# Autodesk Inventor assembly: bubble-wall
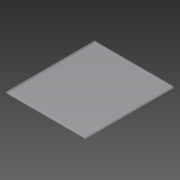
[picture p0: Inventor's stored thumbnail of the model, 180x180]
Saved by Autodesk Inventor 2013 (Build 170138000, 138)
## iProperties
Created: 2013-04-28
Part Number: bubble-wall
Document SubType Name: Assembly
Designer: Chris
Author: Chris
## Documents named in this file (3)
- C:\Users\Chris\Documents\Inventor\Redbull-2013\bubble-wall-final\bubble-wall.iam
- C:\Users\Chris\Documents\Inventor\Redbull-2013\bubble-wall-final\wall-side.ipt
- C:\Users\Chris\Documents\Inventor\Redbull-2013\bubble-wall-final\bottom.ipt
## Components (3 placed, 2 different names)
1. wall-side:1 — Mate:1, Mate:2, Flush:1, Mate:3
2. wall-side:2 — Mate:1, Mate:2, Flush:1, Flush:2, Flush:3
3. bottom:1 — Mate:3, Flush:2, Flush:3
## Relationships (6: Mate 3, Flush 3)
- Mate:1: wall-side:1 ↔ wall-side:2
- Mate:2: wall-side:1 ↔ wall-side:2
- Flush:1: wall-side:1 ↔ wall-side:2
- Mate:3: wall-side:1 ↔ bottom:1
- Flush:2: wall-side:2 ↔ bottom:1
- Flush:3: wall-side:2 ↔ bottom:1
